# Autodesk Inventor assembly: Cryostat top plate
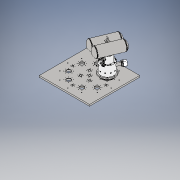
[picture p0: Inventor's stored thumbnail of the model, 180x180]
Saved by Autodesk Inventor 2018 (Build 220112000, 112)
## iProperties
Created: 2018-08-09
Part Number: Cryostat top plate
Document SubType Name: Assembly
Designer: QITI
Author: QITI
## Documents named in this file (4)
- C:\Users\freyja\Documents\Cryorefrigerator\CAD\Cryostat top plate.iam
- C:\Users\freyja\Documents\Cryorefrigerator\CAD\Top Plate.ipt
- C:\Users\freyja\Documents\Cryorefrigerator\CAD\External Models\CH40415 24JUL14 C.ipt
- C:\Users\freyja\Documents\Cryorefrigerator\CAD\vacuum jacket long.ipt
## Components (3 placed, 3 different names)
1. Top Plate:1 — Mate:1, Mate:2, Mate:3, Mate:4, Mate:5, Mate:6
2. CH40415 24JUL14 C:1 — Mate:1, Mate:2, Mate:3
3. vacuum jacket long:1 — Mate:4, Mate:5, Mate:6
## Relationships (6: Mate 6)
- Mate:1: Top Plate:1 ↔ CH40415 24JUL14 C:1
- Mate:2: Top Plate:1 ↔ CH40415 24JUL14 C:1
- Mate:3 (25.4 mm): Top Plate:1 ↔ CH40415 24JUL14 C:1
- Mate:4: Top Plate:1 ↔ vacuum jacket long:1
- Mate:5: Top Plate:1 ↔ vacuum jacket long:1
- Mate:6: Top Plate:1 ↔ vacuum jacket long:1
